# Autodesk Inventor assembly: lados
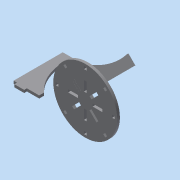
[picture p0: Inventor's stored thumbnail of the model, 180x180]
Saved by Autodesk Inventor 2015 (Build 190159000, 159)
## iProperties
Created: 2017-10-02
Part Number: lados
Document SubType Name: Assembly
Designer: macbook
Author: macbook
## Documents named in this file (3)
- \\Mac\Home\Dropbox\cosplay\espalda\lados\lados.iam
- \\Mac\Home\Dropbox\cosplay\espalda\lados\base.ipt
- \\Mac\Home\Dropbox\cosplay\espalda\lados\brazos.ipt
## Components (3 placed, 2 different names)
1. base:1 — Mate:1, Mate:2, Mate:3
2. brazos:1
3. brazos:2 — Mate:1, Mate:2, Mate:3
## Relationships (3: Mate 3)
- Mate:1: base:1 ↔ brazos:2
- Mate:2: base:1 ↔ brazos:2
- Mate:3: base:1 ↔ brazos:2
